# Autodesk Inventor assembly: z_axys_MIR1
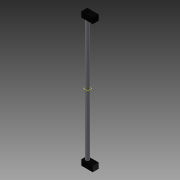
[picture p0: Inventor's stored thumbnail of the model, 180x180]
Saved by Autodesk Inventor 2014 SP1 (Build 180222100, 222)
## iProperties
Created: 2015-04-08
Part Number: z_axys_MIR1
Document SubType Name: Assembly
Designer: Giorgio Nuzzo
Author: Giorgio Nuzzo
## Documents named in this file (4)
- C:\Users\Giorgio Nuzzo\Desktop\3dragmodel\z_axys_MIR1.iam
- C:\Users\Giorgio Nuzzo\Desktop\3dragmodel\supporto_guide_10Z_MIR2.ipt
- C:\Users\Giorgio Nuzzo\Desktop\3dragmodel\guida_Z_MIR1.ipt
- C:\Users\Giorgio Nuzzo\Desktop\3dragmodel\supporto_guide_10Z_MIR_MIR1.ipt
## Components (3 placed, 3 different names)
1. supporto_guide_10Z_MIR2:1 — Mate:1, Flush:1
2. guida_Z_MIR1:1 — Flush:1
3. supporto_guide_10Z_MIR_MIR1:1 — Mate:2
## Relationships (3: Mate 3)
- Mate:1: supporto_guide_10Z_MIR2:1
- Flush:1 [Mate]: supporto_guide_10Z_MIR2:1 ↔ guida_Z_MIR1:1
- Mate:2: supporto_guide_10Z_MIR_MIR1:1
